# Autodesk Inventor assembly: CCM_Unit_D
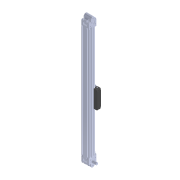
[picture p0: Inventor's stored thumbnail of the model, 180x180]
Saved by Autodesk Inventor 2020 (Build 240168000, 168)
## iProperties
Created: 2021-02-24
Part Number: CCM_Unit_D
Document SubType Name: Assembly
Designer: magnarecta
Author: magnarecta
## Documents named in this file (5)
- D:\Document\Github\Eto_Project\Hardware\Parts\CCM\CCM motion linear guide rail\CCM_UNIT\CCM_Unit_D.iam
- D:\Document\Github\Eto_Project\Hardware\Parts\CCM\CCM motion linear guide rail\CCM_UNIT\TAILSTOCK W40-00_0+0_MIR.ipt
- D:\Document\Github\Eto_Project\Hardware\Parts\CCM\CCM motion linear guide rail\CCM_UNIT\CART HK32-06W-00__1_MIR.ipt
- D:\Document\Github\Eto_Project\Hardware\Parts\CCM\CCM motion linear guide rail\CCM_UNIT\TAILSTOCK W40-00_0+22_1_MIR.ipt
- D:\Document\Github\Eto_Project\Hardware\Parts\CCM\CCM motion linear guide rail\CCM_UNIT\RAIL W40-06_C.ipt
## Components (4 placed, 4 different names)
1. TAILSTOCK W40-00_0+0_MIR:1 — メイト:1, フラッシュ:1, フラッシュ:2, フラッシュ:4
2. CART HK32-06W-00__1_MIR:1 — メイト:3, メイト:4
3. TAILSTOCK W40-00_0+22_1_MIR:1 — メイト:2, フラッシュ:3, フラッシュ:4
4. RAIL W40-06_C:2 — メイト:1, フラッシュ:1, フラッシュ:2, メイト:2, フラッシュ:3, メイト:3, メイト:4
## Relationships (8: Mate 4, Flush 4)
- メイト:1 [Mate]: TAILSTOCK W40-00_0+0_MIR:1 ↔ RAIL W40-06_C:2
- フラッシュ:1 [Flush]: TAILSTOCK W40-00_0+0_MIR:1 ↔ RAIL W40-06_C:2
- フラッシュ:2 [Flush]: TAILSTOCK W40-00_0+0_MIR:1 ↔ RAIL W40-06_C:2
- メイト:2 [Mate]: TAILSTOCK W40-00_0+22_1_MIR:1 ↔ RAIL W40-06_C:2
- フラッシュ:3 [Flush]: TAILSTOCK W40-00_0+22_1_MIR:1 ↔ RAIL W40-06_C:2
- フラッシュ:4 [Flush]: TAILSTOCK W40-00_0+0_MIR:1 ↔ TAILSTOCK W40-00_0+22_1_MIR:1
- メイト:3 [Mate]: CART HK32-06W-00__1_MIR:1 ↔ RAIL W40-06_C:2
- メイト:4 [Mate]: CART HK32-06W-00__1_MIR:1 ↔ RAIL W40-06_C:2
